# Autodesk Inventor assembly: BMG экструдер мой вариант
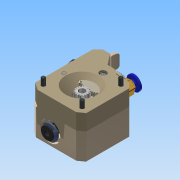
[picture p0: Inventor's stored thumbnail of the model, 180x180]
Saved by Autodesk Inventor 2017 (Build 210142000, 142)
## iProperties
Part Number: BMG экструдер мой вариант
Material: Типовые
Document SubType Name: Assembly
Designer: STALKER
Author: STALKER
## Documents named in this file (18)
- C:\Users\Max\Desktop\Flying Bear Ghost 5\BMG E3DV6 -1.iam
- C:\Users\Max\Desktop\Flying Bear Ghost 5\BMG lower platform.ipt
- C:\Users\Max\Desktop\Flying Bear Ghost 5\MR85 ZZ.ipt
- C:\Users\Max\Desktop\Flying Bear Ghost 5\Adjusting screw.ipt
- C:\Users\Max\Desktop\Flying Bear Ghost 5\Geared gear.ipt
- C:\Users\Max\Desktop\Flying Bear Ghost 5\roller bearing.ipt
- C:\Users\Max\Desktop\Flying Bear Ghost 5\Pinion gear.ipt
- C:\Users\Max\Desktop\Flying Bear Ghost 5\gear rod.ipt
- C:\Users\Max\Desktop\Flying Bear Ghost 5\stock.ipt
- C:\Users\Max\Desktop\Flying Bear Ghost 5\BMG upper platform.ipt
- C:\Users\Max\Desktop\Flying Bear Ghost 5\BMG lever arm.ipt
- C:\Users\Max\Desktop\Flying Bear Ghost 5\m3 nut.ipt
- C:\Users\Max\Desktop\Flying Bear Ghost 5\spring.ipt
- C:\Users\Max\Desktop\Flying Bear Ghost 5\fitting.ipt
- C:\Users\Max\Desktop\Flying Bear Ghost 5\gear motor.ipt
- C:\Users\Max\Desktop\Flying Bear Ghost 5\M3X40.ipt
- C:\Users\Max\Desktop\Flying Bear Ghost 5\fitting E3DV6.ipt
- C:\Users\Max\Desktop\Flying Bear Ghost 5\fitting retainer E3DV6.ipt
## Components (23 placed, 17 different names)
1. BMG lower platform:1 — Совмещение:1, Совмещение:2, Совмещение:4, Заподлицо:1, Совмещение:5, Совмещение:6, Совмещение:7, Совмещение:8, Совмещение:9, Совмещение:16, Заподлицо:5, Угол:1, Угол:2, Совмещение:21, Совмещение:22, Заподлицо:6, Совмещение:27, Совмещение:28, Совмещение:37, Совмещение:38, Совмещение:39, Заподлицо:10
2. MR85 ZZ:1 — Совмещение:1, Совмещение:2
3. Adjusting screw:1 — Совмещение:18, Совмещение:19, Совмещение:22, Заподлицо:6, Совмещение:23, Совмещение:24
4. Geared gear:1 — Совмещение:3, Совмещение:4, Совмещение:5
5. roller bearing:1 — Совмещение:11, Совмещение:12, Заподлицо:2
6. Pinion gear:1 — Совмещение:3, Заподлицо:1
7. gear rod:1 — Совмещение:10, Совмещение:11, Совмещение:13, Совмещение:14, Заподлицо:3
8. stock:1 — Совмещение:15, Совмещение:16, Заподлицо:4
9. Pinion gear:2 — Заподлицо:2, Совмещение:13, Заподлицо:5
10. BMG upper platform:1 — Совмещение:6, Совмещение:7, Совмещение:8, Заподлицо:4, Совмещение:17, Совмещение:25, Совмещение:26, Совмещение:40, Совмещение:43
11. BMG lever arm:1 — Совмещение:9, Совмещение:14, Заподлицо:3, Совмещение:15, Совмещение:17
12. roller bearing:2 — Совмещение:10, Совмещение:12
13. m3 nut:1 — Совмещение:18, Совмещение:20, Угол:1, Совмещение:21
14. m3 nut:2 — Совмещение:19, Совмещение:20, Угол:2
15. spring:1 — Совмещение:23, Совмещение:24
16. MR85 ZZ:2 — Совмещение:25, Совмещение:26
17. fitting:1 — Совмещение:27, Совмещение:28
18. gear motor:1
19. M3X40:1 — Совмещение:37, Заподлицо:8
20. M3X40:2 — Совмещение:38, Заподлицо:9, Заподлицо:10
21. M3X40:3 — Совмещение:39, Заподлицо:8, Заподлицо:9
22. fitting E3DV6:1 — Совмещение:40, Совмещение:41, Совмещение:42
23. fitting retainer E3DV6:1 — Совмещение:41, Совмещение:42, Совмещение:43
## Relationships (46: Mate 35, Flush 9, Angle 2)
- Совмещение:1 [Mate]: BMG lower platform:1 ↔ MR85 ZZ:1
- Совмещение:2 [Mate]: BMG lower platform:1 ↔ MR85 ZZ:1
- Совмещение:3 [Mate]: Geared gear:1 ↔ Pinion gear:1
- Совмещение:4 [Mate]: BMG lower platform:1 ↔ Geared gear:1
- Заподлицо:1 [Flush]: BMG lower platform:1 ↔ Pinion gear:1
- Совмещение:5 [Mate]: BMG lower platform:1 ↔ Geared gear:1
- Совмещение:6 [Mate]: BMG lower platform:1 ↔ BMG upper platform:1
- Совмещение:7 [Mate]: BMG lower platform:1 ↔ BMG upper platform:1
- Совмещение:8 [Mate]: BMG lower platform:1 ↔ BMG upper platform:1
- Совмещение:9 [Mate]: BMG lower platform:1 ↔ BMG lever arm:1
- Совмещение:10 [Mate]: gear rod:1 ↔ roller bearing:2
- Совмещение:11 [Mate]: roller bearing:1 ↔ gear rod:1
- Совмещение:12 [Mate]: roller bearing:1 ↔ roller bearing:2
- Заподлицо:2 [Flush]: roller bearing:1 ↔ Pinion gear:2
- Совмещение:13 [Mate]: gear rod:1 ↔ Pinion gear:2
- Совмещение:14 [Mate]: gear rod:1 ↔ BMG lever arm:1
- Заподлицо:3 [Flush]: gear rod:1 ↔ BMG lever arm:1
- Совмещение:15 [Mate]: stock:1 ↔ BMG lever arm:1
- Совмещение:16 [Mate]: BMG lower platform:1 ↔ stock:1
- Заподлицо:4 [Flush]: stock:1 ↔ BMG upper platform:1
- Совмещение:17 [Mate] (0.2 mm): BMG upper platform:1 ↔ BMG lever arm:1
- Заподлицо:5 [Flush]: BMG lower platform:1 ↔ Pinion gear:2
- Совмещение:18 [Mate]: Adjusting screw:1 ↔ m3 nut:1
- Совмещение:19 [Mate]: Adjusting screw:1 ↔ m3 nut:2
- Совмещение:20 [Mate]: m3 nut:1 ↔ m3 nut:2
- Угол:1 [Angle] (0 deg): BMG lower platform:1 ↔ m3 nut:1
- Угол:2 [Angle] (0 deg): BMG lower platform:1 ↔ m3 nut:2
- Совмещение:21 [Mate]: BMG lower platform:1 ↔ m3 nut:1
- Совмещение:22 [Mate]: BMG lower platform:1 ↔ Adjusting screw:1
- Заподлицо:6 [Flush] (-20 mm): BMG lower platform:1 ↔ Adjusting screw:1
- Совмещение:23 [Mate]: Adjusting screw:1 ↔ spring:1
- Совмещение:24 [Mate]: Adjusting screw:1 ↔ spring:1
- Совмещение:25 [Mate]: BMG upper platform:1 ↔ MR85 ZZ:2
- Совмещение:26 [Mate]: BMG upper platform:1 ↔ MR85 ZZ:2
- Совмещение:27 [Mate]: BMG lower platform:1 ↔ fitting:1
- Совмещение:28 [Mate]: BMG lower platform:1 ↔ fitting:1
- Совмещение:37 [Mate]: BMG lower platform:1 ↔ M3X40:1
- Совмещение:38 [Mate]: BMG lower platform:1 ↔ M3X40:2
- Совмещение:39 [Mate]: BMG lower platform:1 ↔ M3X40:3
- Заподлицо:8 [Flush]: M3X40:1 ↔ M3X40:3
- Заподлицо:9 [Flush]: M3X40:2 ↔ M3X40:3
- Заподлицо:10 [Flush]: BMG lower platform:1 ↔ M3X40:2
- Совмещение:40 [Mate]: BMG upper platform:1 ↔ fitting E3DV6:1
- Совмещение:41 [Mate]: fitting E3DV6:1 ↔ fitting retainer E3DV6:1
- Совмещение:42 [Mate]: fitting E3DV6:1 ↔ fitting retainer E3DV6:1
- Совмещение:43 [Mate]: BMG upper platform:1 ↔ fitting retainer E3DV6:1
